# Autodesk Inventor assembly: load_cell_holder_assembly
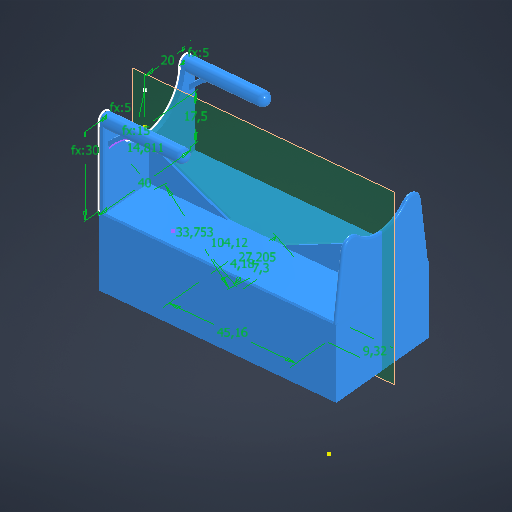
[picture p0: Inventor's stored thumbnail of the model, 512x512]
Saved by Autodesk Inventor 2026 (Build 300175000, 175)
## iProperties
Created: 2025-04-22
Part Number: load_cell_holder_assembly
Document SubType Name: Assembly
Designer: Paul Juschitz
Author: Paul Juschitz
## Documents named in this file (3)
- C:\Users\Paul Juschitz\Documents\private\m5_GBW_mod\M5_GBW_mod\CAD\load_cell_holder_assembly.iam
- C:\Users\Paul Juschitz\Documents\private\m5_GBW_mod\M5_GBW_mod\CAD\load_cell_dowel_pin_screw.iam
- C:\Users\Paul Juschitz\Documents\private\m5_GBW_mod\M5_GBW_mod\CAD\my_portafilter_holder_5.ipt
## Components (2 placed, 2 different names)
1. load_cell_dowel_pin_screw:1 [sub-assembly] — Cylindrical:1, Angle:1, Mate:1
2. my_portafilter_holder_5:1 — Cylindrical:1, Angle:1, Mate:1
## Relationships (3: CylindricalJoint 1, Angle 1, Mate 1)
- Cylindrical:1: load_cell_dowel_pin_screw:1 ↔ my_portafilter_holder_5:1
- Angle:1 (180 deg): load_cell_dowel_pin_screw:1 ↔ my_portafilter_holder_5:1
- Mate:1: load_cell_dowel_pin_screw:1 ↔ my_portafilter_holder_5:1
